# Autodesk Inventor assembly: ASY GBK центральная стенка
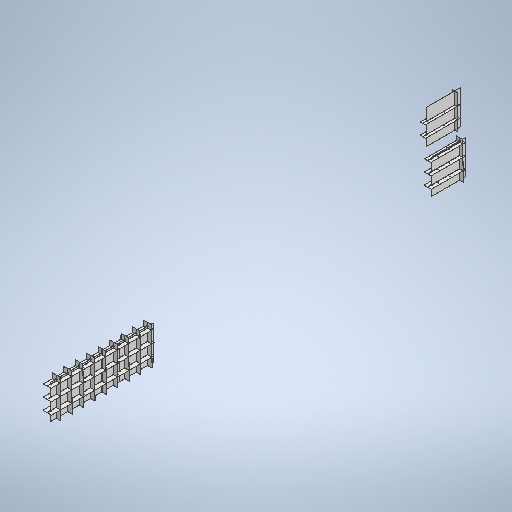
[picture p0: Inventor's stored thumbnail of the model, 512x512]
Saved by Autodesk Inventor 2026 (Build 300175000, 175)
## iProperties
Created: 2026-05-28
Part Number: ASY GBK центральная стенка
Document SubType Name: Assembly
Designer: pokla
Author: pokla
## Documents named in this file (5)
- C:\Users\pokla\Documents\Inventor\GBK-Gubkinskiy\ASY GBK центральная стенка.iam
- C:\Users\pokla\Documents\Inventor\GBK-Gubkinskiy\ASY GBK 3210 wall shield Center 3.iam
- C:\Users\pokla\Documents\Inventor\GBK-Gubkinskiy\ASY GBK 3310 wall shield Center 4.iam
- C:\Users\pokla\Documents\Inventor\GBK-Gubkinskiy\ASY GBK 3110 central wall shield 1.iam
- C:\Users\pokla\Documents\Inventor\GBK-Gubkinskiy\ASY GBK 3120 central wall shield 2.iam
## Components (4 placed, 4 different names)
1. ASY GBK 3310 wall shield Center 4.iam:1 [sub-assembly]
2. ASY GBK 3210 wall shield Center 3.iam:1 [sub-assembly]
3. ASY GBK 3110 central wall shield 1:1 [sub-assembly] — Совмещение:1, Совмещение:3, Жесткий:1, Совмещение:4
4. ASY GBK 3120 central wall shield 2:1 [sub-assembly] — Жесткий:1
## Relationships (4: Mate 3, WeldJoint 1)
- Совмещение:1 [Mate]: ASY GBK 3110 central wall shield 1:1
- Совмещение:3 [Mate]: ASY GBK 3110 central wall shield 1:1
- Жесткий:1 [WeldJoint] (1 mm): ASY GBK 3110 central wall shield 1:1 ↔ ASY GBK 3120 central wall shield 2:1
- Совмещение:4 [Mate]: ASY GBK 3110 central wall shield 1:1
